# Autodesk Inventor assembly: element_L
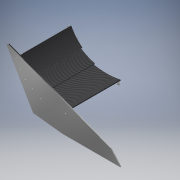
[picture p0: Inventor's stored thumbnail of the model, 180x180]
Saved by Autodesk Inventor 2018.1 (Build 221171000, 171)
## iProperties
Created: 2017-10-22
Part Number: element_L
Material: 一般
Document SubType Name: Assembly
Designer: ku_sk
Author: ku_sk
## Documents named in this file (5)
- D:\ku_sk\ドキュメント\Inventor\KS-15_Aero_CAD\type4\F-wing\parts\element_side\element_L.iam
- D:\ku_sk\ドキュメント\Inventor\KS-15_Aero_CAD\type4\F-wing\parts\element_side\parts\element_1.ipt
- D:\ku_sk\ドキュメント\Inventor\KS-15_Aero_CAD\type4\F-wing\parts\element_side\parts\element_2.ipt
- D:\ku_sk\ドキュメント\Inventor\KS-15_Aero_CAD\type4\F-wing\parts\element_clip.ipt
- D:\ku_sk\ドキュメント\Inventor\KS-15_Aero_CAD\type4\F-wing\parts\element_side\parts\stay_middle.ipt
## Components (16 placed, 4 different names)
1. stay_middle:1 — フラッシュ:18, フラッシュ:19, メイト:24, メイト:25, メイト:26, メイト:27, メイト:28, メイト:29, フラッシュ:20
2. element_1:1 — メイト:13, メイト:14, フラッシュ:13, フラッシュ:14, メイト:15, メイト:16, メイト:17, メイト:18, フラッシュ:15, フラッシュ:16, メイト:19, メイト:20
3. element_2:1 — フラッシュ:1, メイト:1, フラッシュ:2, メイト:3, フラッシュ:5, フラッシュ:6, メイト:5, フラッシュ:10, メイト:8, メイト:9, フラッシュ:11, メイト:11
4. element_2:2 — メイト:2, フラッシュ:3, フラッシュ:4, メイト:4, フラッシュ:7, フラッシュ:8, メイト:6, フラッシュ:9, メイト:7, メイト:10, フラッシュ:12, メイト:12
5. element_clip:1 — フラッシュ:1, メイト:1, フラッシュ:2
6. element_clip:2 — メイト:2, フラッシュ:3, フラッシュ:4
7. element_clip:3 — メイト:5, フラッシュ:10, メイト:8, メイト:27
8. element_clip:4 — メイト:6, フラッシュ:9, メイト:7, メイト:28
9. element_clip:5 — メイト:13, フラッシュ:13, メイト:16
10. element_clip:6 — メイト:14, フラッシュ:14, メイト:15, メイト:29
11. element_clip:7 — メイト:3, フラッシュ:5, フラッシュ:6
12. element_clip:8 — メイト:4, フラッシュ:7, フラッシュ:8
13. element_clip:9 — メイト:9, フラッシュ:11, メイト:11, メイト:24
14. element_clip:10 — メイト:10, フラッシュ:12, メイト:12, メイト:25
15. element_clip:11 — メイト:17, フラッシュ:15, メイト:20
16. element_clip:12 — メイト:18, フラッシュ:16, メイト:19, メイト:26
## Relationships (45: Mate 26, Flush 19)
- フラッシュ:1 [Flush]: element_2:1 ↔ element_clip:1
- メイト:1 [Mate]: element_2:1 ↔ element_clip:1
- フラッシュ:2 [Flush]: element_2:1 ↔ element_clip:1
- メイト:2 [Mate]: element_2:2 ↔ element_clip:2
- フラッシュ:3 [Flush]: element_2:2 ↔ element_clip:2
- フラッシュ:4 [Flush]: element_2:2 ↔ element_clip:2
- メイト:3 [Mate]: element_2:1 ↔ element_clip:7
- メイト:4 [Mate]: element_2:2 ↔ element_clip:8
- フラッシュ:5 [Flush]: element_2:1 ↔ element_clip:7
- フラッシュ:6 [Flush]: element_2:1 ↔ element_clip:7
- フラッシュ:7 [Flush]: element_2:2 ↔ element_clip:8
- フラッシュ:8 [Flush]: element_2:2 ↔ element_clip:8
- メイト:5 [Mate]: element_2:1 ↔ element_clip:3
- メイト:6 [Mate]: element_2:2 ↔ element_clip:4
- フラッシュ:9 [Flush]: element_2:2 ↔ element_clip:4
- メイト:7 [Mate]: element_2:2 ↔ element_clip:4
- フラッシュ:10 [Flush]: element_2:1 ↔ element_clip:3
- メイト:8 [Mate]: element_2:1 ↔ element_clip:3
- メイト:9 [Mate]: element_2:1 ↔ element_clip:9
- メイト:10 [Mate]: element_2:2 ↔ element_clip:10
- フラッシュ:11 [Flush]: element_2:1 ↔ element_clip:9
- メイト:11 [Mate]: element_2:1 ↔ element_clip:9
- フラッシュ:12 [Flush]: element_2:2 ↔ element_clip:10
- メイト:12 [Mate]: element_2:2 ↔ element_clip:10
- メイト:13 [Mate]: element_1:1 ↔ element_clip:5
- メイト:14 [Mate]: element_1:1 ↔ element_clip:6
- フラッシュ:13 [Flush]: element_1:1 ↔ element_clip:5
- フラッシュ:14 [Flush]: element_1:1 ↔ element_clip:6
- メイト:15 [Mate]: element_1:1 ↔ element_clip:6
- メイト:16 [Mate]: element_1:1 ↔ element_clip:5
- メイト:17 [Mate]: element_1:1 ↔ element_clip:11
- メイト:18 [Mate]: element_1:1 ↔ element_clip:12
- フラッシュ:15 [Flush]: element_1:1 ↔ element_clip:11
- フラッシュ:16 [Flush]: element_1:1 ↔ element_clip:12
- メイト:19 [Mate]: element_1:1 ↔ element_clip:12
- メイト:20 [Mate]: element_1:1 ↔ element_clip:11
- フラッシュ:18 [Flush]: stay_middle:1
- フラッシュ:19 [Flush]: stay_middle:1
- メイト:24 [Mate]: stay_middle:1 ↔ element_clip:9
- メイト:25 [Mate]: stay_middle:1 ↔ element_clip:10
- メイト:26 [Mate]: stay_middle:1 ↔ element_clip:12
- メイト:27 [Mate]: stay_middle:1 ↔ element_clip:3
- メイト:28 [Mate]: stay_middle:1 ↔ element_clip:4
- メイト:29 [Mate]: stay_middle:1 ↔ element_clip:6
- フラッシュ:20 [Flush]: stay_middle:1
